# Autodesk Inventor assembly: Batteriepack
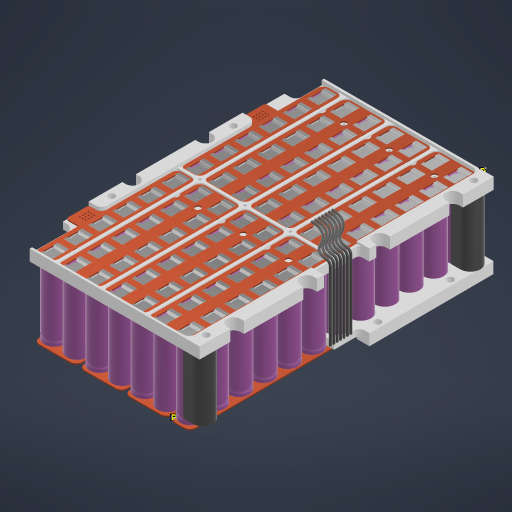
[picture p0: Inventor's stored thumbnail of the model, 512x512]
Saved by Autodesk Inventor 2024.3 (Build 283343010, 343A)
## iProperties
Created: 2025-03-26
Part Number: Batteriepack
Document SubType Name: Assembly
Designer: David Lill
Author: David Lill
## Documents named in this file (11)
- C:\Users\David\Documents\FTAG\E-16\Batterie\Batterie_Konstruktion\E-16 Batterie\Batteriepack.iam
- C:\Users\David\Documents\FTAG\E-16\Batterie\Batterie_Konstruktion\E-16 Batterie\Platte1.ipt
- C:\Users\David\Documents\FTAG\E-16\Batterie\Batterie_Konstruktion\E-16 Batterie\Abstandhalter.ipt
- C:\Users\David\Documents\FTAG\E-16\Batterie\Batterie_Konstruktion\E-16 Batterie\Bat_contacts_v2.iam
- C:\Users\David\Documents\FTAG\E-16\Batterie\Batterie_Konstruktion\E-16 Batterie\18650_assembly.iam
- C:\Users\David\Documents\FTAG\E-16\Batterie\Batterie_Konstruktion\E-16 Batterie\Bat_contacts_v2_long.iam
- C:\Users\David\Documents\FTAG\E-16\Batterie\Batterie_Konstruktion\E-16 Batterie\Bat_contacts_v2_contact.iam
- C:\Users\David\Documents\FTAG\E-16\Batterie\Batterie_Konstruktion\E-16 Batterie\Platte2.ipt
- C:\Users\David\Documents\FTAG\E-16\Batterie\Batterie_Konstruktion\E-16 Batterie\Bat_contacts_v2_contact_mir.iam
- C:\Users\David\Documents\FTAG\E-16\Batterie\Batterie_Konstruktion\E-16 Batterie\Kabelstrang.ipt
- C:\Users\David\Documents\FTAG\E-16\Batterie\Batterie_Konstruktion\E-16 Batterie\Batteriepack\AIP\Kabel und Kabelbaum\Batteriepack.Kabelbaum1.iam
## Components (24 placed, 10 different names)
1. Platte1:4 — Einfügen:11, Einfügen:12, Einfügen:13, Einfügen:16, Fluchtend:1, Passend:11, Passend:17, Passend:19, Passend:21, Einfügen:18, Passend:23, Passend:33, Passend:35, Passend:36, Passend:37
2. Abstandhalter:1 — Einfügen:12
3. Abstandhalter:2 — Einfügen:11, Passend:25, Passend:30
4. 18650_assembly:1 [sub-assembly] — Einfügen:13, Einfügen:16, Passend:6, Passend:7, Passend:10, Einfügen:17, Passend:22, Passend:24, Passend:30, Passend:31, Passend:32
5. Bat_contacts_v2_long:1 [sub-assembly] — Passend:6, Passend:28, Passend:29
6. Bat_contacts_v2_contact:1 [sub-assembly] — Passend:10, Passend:11, Passend:36
7. Platte2:1 — Einfügen:17, Passend:21, Passend:25, Passend:26, Passend:27, Passend:28, Passend:29
8. Abstandhalter:3 — Einfügen:18, Passend:22
9. Abstandhalter:4 — Passend:23, Passend:24
10. Bat_contacts_v2_contact_mir:1 [sub-assembly] — Passend:32, Passend:33, Passend:37
11. Kabelstrang:1
12. Kabelbaum1 [sub-assembly]
13. Bat_contacts_v2:1 [sub-assembly] — Fluchtend:1, Passend:31
14. Bat_contacts_v2:7 [sub-assembly] — Passend:7, Passend:26, Passend:27
15. Bat_contacts_v2:2 [sub-assembly]
16. Bat_contacts_v2:8 [sub-assembly]
17. Bat_contacts_v2:3 [sub-assembly]
18. Bat_contacts_v2:9 [sub-assembly]
19. Bat_contacts_v2:4 [sub-assembly]
20. Bat_contacts_v2:10 [sub-assembly]
21. Bat_contacts_v2:5 [sub-assembly]
22. Bat_contacts_v2:11 [sub-assembly]
23. Bat_contacts_v2:6 [sub-assembly] — Passend:35
24. Bat_contacts_v2:12 [sub-assembly]
## Component patterns: (6 elements, first: Bat_contacts_v2:1 + Bat_contacts_v2:7)
## Relationships (29: Mate 22, Insert 6, Flush 1)
- Einfügen:11 [Insert]: Platte1:4 ↔ Abstandhalter:2
- Einfügen:12 [Insert]: Platte1:4 ↔ Abstandhalter:1
- Einfügen:13 [Insert]: Platte1:4 ↔ 18650_assembly:1
- Einfügen:16 [Insert]: Platte1:4 ↔ 18650_assembly:1
- Fluchtend:1 [Flush] (2 mm): Platte1:4 ↔ Bat_contacts_v2:1
- Passend:6 [Mate]: 18650_assembly:1 ↔ Bat_contacts_v2_long:1
- Passend:7 [Mate]: 18650_assembly:1 ↔ Bat_contacts_v2:7
- Passend:10 [Mate]: 18650_assembly:1 ↔ Bat_contacts_v2_contact:1
- Passend:11 [Mate]: Platte1:4 ↔ Bat_contacts_v2_contact:1
- Passend:17 [Mate] (-130 mm): Platte1:4
- Passend:19 [Mate]: Platte1:4
- Einfügen:17 [Insert]: 18650_assembly:1 ↔ Platte2:1
- Passend:21 [Mate]: Platte1:4 ↔ Platte2:1
- Einfügen:18 [Insert]: Platte1:4 ↔ Abstandhalter:3
- Passend:22 [Mate]: 18650_assembly:1 ↔ Abstandhalter:3
- Passend:23 [Mate]: Platte1:4 ↔ Abstandhalter:4
- Passend:24 [Mate]: 18650_assembly:1 ↔ Abstandhalter:4
- Passend:25 [Mate]: Abstandhalter:2 ↔ Platte2:1
- Passend:26 [Mate]: Platte2:1 ↔ Bat_contacts_v2:7
- Passend:27 [Mate]: Platte2:1 ↔ Bat_contacts_v2:7
- Passend:28 [Mate]: Bat_contacts_v2_long:1 ↔ Platte2:1
- Passend:29 [Mate]: Bat_contacts_v2_long:1 ↔ Platte2:1
- Passend:30 [Mate]: Abstandhalter:2 ↔ 18650_assembly:1
- Passend:31 [Mate]: 18650_assembly:1 ↔ Bat_contacts_v2:1
- Passend:32 [Mate]: 18650_assembly:1 ↔ Bat_contacts_v2_contact_mir:1
- Passend:33 [Mate]: Platte1:4 ↔ Bat_contacts_v2_contact_mir:1
- Passend:35 [Mate]: Platte1:4 ↔ Bat_contacts_v2:6
- Passend:36 [Mate]: Platte1:4 ↔ Bat_contacts_v2_contact:1
- Passend:37 [Mate]: Platte1:4 ↔ Bat_contacts_v2_contact_mir:1
